# Autodesk Inventor assembly: MAIN_MODULE
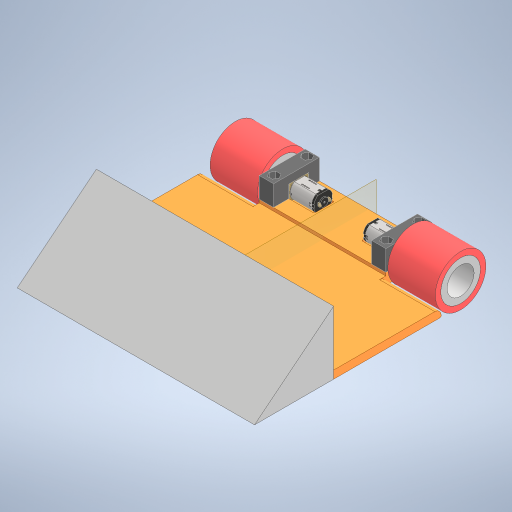
[picture p0: Inventor's stored thumbnail of the model, 512x512]
Saved by Autodesk Inventor 2023 (Build 270158000, 158)
## iProperties
Created: 2024-04-04
Part Number: MAIN_MODULE
Document SubType Name: Assembly
Designer: Kamil
Author: Kamil
## Documents named in this file (9)
- C:\Users\Kamil\Documents\PROJEKT ZESPOLOWY\mechanics\MAIN_MODULE.iam
- C:\Users\Kamil\Documents\PROJEKT ZESPOLOWY\mechanics\STEP\N20 DC MOTOR.ipt
- C:\Users\Kamil\Documents\PROJEKT ZESPOLOWY\mechanics\base.ipt
- C:\Users\Kamil\Documents\PROJEKT ZESPOLOWY\mechanics\kolo.ipt
- C:\Users\Kamil\Documents\PROJEKT ZESPOLOWY\mechanics\tire.ipt
- C:\Users\Kamil\Documents\PROJEKT ZESPOLOWY\mechanics\motor_bracket.ipt
- C:\Users\Kamil\Documents\PROJEKT ZESPOLOWY\mechanics\motor_bracket_MIR.ipt
- C:\Users\Kamil\Documents\PROJEKT ZESPOLOWY\mechanics\sumo_module_shield.ipt
- C:\Users\Kamil\Documents\PROJEKT ZESPOLOWY\mechanics\TOF_VL53L0X (1).ipt
## Components (12 placed, 8 different names)
1. N20 DC MOTOR:1 — Równoległe:1, Zestawiające:3, Zestawiające:6, Zestawiające:9, Równoległe:3, Kątowe:1
2. N20 DC MOTOR:2 — Równoległe:2, Zestawiające:3, Zestawiające:7, Zestawiające:8, Kątowe:2, Równoległe:7
3. base:1 — Równoległe:1, Równoległe:2, Równoległe:3, Zestawiające:13, Równoległe:6, Symetria:1, Równoległe:8, Równoległe:9, Zestawiające:14
4. kolo:1 — Zestawiające:6, Zestawiające:9, Równoległe:4, Zestawiające:12, Kątowe:1
5. kolo:2 — Zestawiające:7, Zestawiające:8, Równoległe:5, Zestawiające:11, Kątowe:2
6. tire:1 — Równoległe:4, Zestawiające:12
7. tire:2 — Równoległe:5, Zestawiające:11
8. motor_bracket:1 — Zestawiające:13, Równoległe:6, Równoległe:7, Symetria:1
9. motor_bracket_MIR:1
10. sumo_module_shield:1 — Równoległe:8, Równoległe:9, Zestawiające:14, Zestawiające:15, Zestawiające:16, Równoległe:10, Równoległe:11
11. TOF_VL53L0X (1):1 — Zestawiające:16, Równoległe:10
12. TOF_VL53L0X (1):2 — Zestawiające:15, Równoległe:11
## Relationships (25: Flush 11, Mate 11, Angle 2, Symmetry 1)
- Równoległe:1 [Flush]: N20 DC MOTOR:1 ↔ base:1
- Równoległe:2 [Flush]: N20 DC MOTOR:2 ↔ base:1
- Zestawiające:3 [Mate]: N20 DC MOTOR:1 ↔ N20 DC MOTOR:2
- Zestawiające:6 [Mate] (0.5 mm): N20 DC MOTOR:1 ↔ kolo:1
- Zestawiające:7 [Mate] (0.5 mm): N20 DC MOTOR:2 ↔ kolo:2
- Zestawiające:8 [Mate]: N20 DC MOTOR:2 ↔ kolo:2
- Zestawiające:9 [Mate]: N20 DC MOTOR:1 ↔ kolo:1
- Równoległe:3 [Flush] (-5 mm): N20 DC MOTOR:1 ↔ base:1
- Równoległe:4 [Flush]: kolo:1 ↔ tire:1
- Równoległe:5 [Flush]: kolo:2 ↔ tire:2
- Zestawiające:11 [Mate]: kolo:2 ↔ tire:2
- Zestawiające:12 [Mate]: kolo:1 ↔ tire:1
- Kątowe:1 [Angle] (180 deg): N20 DC MOTOR:1 ↔ kolo:1
- Kątowe:2 [Angle] (180 deg): N20 DC MOTOR:2 ↔ kolo:2
- Zestawiające:13 [Mate]: base:1 ↔ motor_bracket:1
- Równoległe:6 [Flush]: base:1 ↔ motor_bracket:1
- Równoległe:7 [Flush]: N20 DC MOTOR:2 ↔ motor_bracket:1
- Symetria:1 [Symmetry]: base:1 ↔ motor_bracket:1
- Równoległe:8 [Flush]: base:1 ↔ sumo_module_shield:1
- Równoległe:9 [Flush]: base:1 ↔ sumo_module_shield:1
- Zestawiające:14 [Mate]: base:1 ↔ sumo_module_shield:1
- Zestawiające:15 [Mate]: sumo_module_shield:1 ↔ TOF_VL53L0X (1):2
- Zestawiające:16 [Mate]: sumo_module_shield:1 ↔ TOF_VL53L0X (1):1
- Równoległe:10 [Flush] (-10 mm): sumo_module_shield:1 ↔ TOF_VL53L0X (1):1
- Równoległe:11 [Flush] (-10 mm): sumo_module_shield:1 ↔ TOF_VL53L0X (1):2
